# Autodesk Inventor assembly: modelo cad brazo
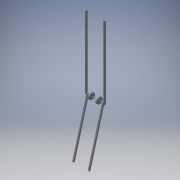
[picture p0: Inventor's stored thumbnail of the model, 180x180]
Saved by Autodesk Inventor 2016 (Build 200138000, 138)
## iProperties
Created: 2016-07-27
Part Number: modelo cad brazo
Document SubType Name: Assembly
Designer: Admin
Author: Admin
## Documents named in this file (4)
- C:\Users\Admin\Documents\diseños autodesk dimer\engranajes dimer hombro muelles\modelo cad brazo.iam
- C:\Users\Admin\Documents\diseños autodesk dimer\engranajes dimer hombro muelles\modelo cad brazo.ipt
- C:\Users\Admin\Documents\diseños autodesk dimer\engranajes dimer hombro muelles\antebrazo.ipt
- C:\Users\Admin\Documents\diseños autodesk dimer\engranajes dimer hombro muelles\rodamientos medio.ipt
## Components (4 placed, 3 different names)
1. modelo cad brazo:1 — Mate:1, Mate:2
2. antebrazo:1 — Mate:1, Mate:2, Mate:3, Mate:4
3. rodamientos medio:1 — Mate:3
4. rodamientos medio:2 — Mate:4
## Relationships (4: Mate 4)
- Mate:1 (0.75 mm): modelo cad brazo:1 ↔ antebrazo:1
- Mate:2: modelo cad brazo:1 ↔ antebrazo:1
- Mate:3: antebrazo:1 ↔ rodamientos medio:1
- Mate:4: antebrazo:1 ↔ rodamientos medio:2
